# Autodesk Inventor assembly: Belt Tensioner 10mm
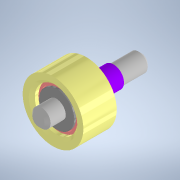
[picture p0: Inventor's stored thumbnail of the model, 180x180]
Saved by Autodesk Inventor 2022.2 (Build 262287000, 287)
## iProperties
Created: 2022-01-06
Part Number: Belt Tensioner 10mm
Document SubType Name: Assembly
Designer: Jochen
Author: Jochen
## Documents named in this file (6)
- D:\Projects\Chewbacca\CAD\Common\Belt Tensioner\BeltTensioner 10mm.iam
- D:\Projects\Chewbacca\CAD\Common\Belt Tensioner\BeltTensionerRoller 10mm.ipt
- D:\Projects\Chewbacca\CAD\Common\Bearing\bearing_7_3_3_sbn_683_2ZVA.ipt
- D:\Projects\Chewbacca\CAD\Common\Washer\Washer m2.5.ipt
- D:\Projects\Chewbacca\CAD\Common\Belt Tensioner\MotorBeltTensionerAxis.ipt
- D:\Projects\Chewbacca\CAD\Common\Belt Tensioner\OutputBeltTensionerSleeve 5mm.ipt
## Components (5 placed, 5 different names)
1. Belt Tensioner 10mm:1 — Mate:18, Mate:19, Mate:22
2. bearing_7_3_3_sbn_683_2ZVA:1 — Mate:9, Mate:18, Mate:19, Mate:20, Mate:24
3. Washer m2.5:1 — Mate:9, Mate:21, Mate:22
4. MotorBeltTensionerAxis:1 — Mate:20, Mate:21, Mate:23
5. OutputBeltTensionerSleeve 6mm:1 — Mate:23, Mate:24
## Relationships (8: Mate 8)
- Mate:9: bearing_7_3_3_sbn_683_2ZVA:1 ↔ Washer m2.5:1
- Mate:18: Belt Tensioner 10mm:1 ↔ bearing_7_3_3_sbn_683_2ZVA:1
- Mate:19: Belt Tensioner 10mm:1 ↔ bearing_7_3_3_sbn_683_2ZVA:1
- Mate:20: bearing_7_3_3_sbn_683_2ZVA:1 ↔ MotorBeltTensionerAxis:1
- Mate:21 (3 mm): Washer m2.5:1 ↔ MotorBeltTensionerAxis:1
- Mate:22: Belt Tensioner 10mm:1 ↔ Washer m2.5:1
- Mate:23: MotorBeltTensionerAxis:1 ↔ OutputBeltTensionerSleeve 6mm:1
- Mate:24: bearing_7_3_3_sbn_683_2ZVA:1 ↔ OutputBeltTensionerSleeve 6mm:1
